# Autodesk Inventor assembly: bay con 12 mk2
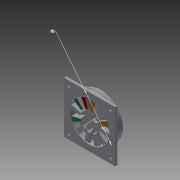
[picture p0: Inventor's stored thumbnail of the model, 180x180]
Saved by Autodesk Inventor 2015 (Build 190159000, 159)
## iProperties
Created: 2014-10-24
Part Number: bay con 12 mk2
Document SubType Name: Assembly
Designer: ericd_000
Author: ericd_000
## Documents named in this file (3)
- C:\Users\ericd_000\Dropbox\GitHub\initial_cad\eric_cad\bay con 12 mk2.iam
- C:\Users\ericd_000\Dropbox\GitHub\initial_cad\eric_cad\bayonet container 12.ipt
- C:\Users\ericd_000\Dropbox\GitHub\initial_cad\eric_cad\inner bayonet connector 12.ipt
## Components (2 placed, 2 different names)
1. bayonet container 12:1 — Cylindrical:1, Cylindrical:2
2. inner bayonet connector 12:1 — Cylindrical:1, Cylindrical:2
## Relationships (2: CylindricalJoint 2)
- Cylindrical:1: bayonet container 12:1 ↔ inner bayonet connector 12:1
- Cylindrical:2: bayonet container 12:1 ↔ inner bayonet connector 12:1
